# Autodesk Inventor assembly: Robot_V1.0
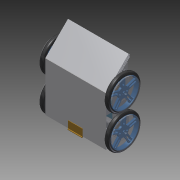
[picture p0: Inventor's stored thumbnail of the model, 180x180]
Saved by Autodesk Inventor 2013 (Build 170138000, 138)
## iProperties
Created: 2015-07-02
Part Number: Robot_V1.0
Document SubType Name: Assembly
Designer: Kyle
Mass: 370.984 g
Surface Area: 2505.11 cm^2
Volume: 171.813 cm^3
Density: 2.15924 g/cm^3
Author: Kyle
## Documents named in this file (16)
- C:\Users\Kyle\Documents\Project documentation\Combat Robot\CAD\V1.0\Robot_V1.0.iam
- C:\Users\Kyle\Documents\Project documentation\Combat Robot\CAD\V1.0\Armor_Rear.iam
- C:\Users\Kyle\Documents\Project documentation\Combat Robot\CAD\V1.0\Armor_Front.iam
- C:\Users\Kyle\Documents\Project documentation\Combat Robot\CAD\V1.0\Gearmotor.iam
- C:\Users\Kyle\Documents\Project documentation\Combat Robot\CAD\V1.0\LiPo.ipt
- C:\Users\Kyle\Documents\Project documentation\Combat Robot\CAD\V1.0\Rx.ipt
- C:\Users\Kyle\Documents\Project documentation\Combat Robot\CAD\V1.0\Plate_InnerSide_Poly.ipt
- C:\Users\Kyle\Documents\Project documentation\Combat Robot\CAD\V1.0\Reinforcer_Front.ipt
- C:\Users\Kyle\Documents\Project documentation\Combat Robot\CAD\V1.0\Bracket.ipt
- C:\Users\Kyle\Documents\Project documentation\Combat Robot\CAD\V1.0\Hinge_Rear.ipt
- C:\Users\Kyle\Documents\Project documentation\Combat Robot\CAD\V1.0\Wheel_60mm.iam
- C:\Users\Kyle\Documents\Project documentation\Combat Robot\CAD\V1.0\Mount_Motor.ipt
- C:\Users\Kyle\Documents\Project documentation\Combat Robot\CAD\V1.0\Bracket_Motor.ipt
- C:\Users\Kyle\Documents\Project documentation\Combat Robot\CAD\V1.0\Plate_Wheel.ipt
- C:\Users\Kyle\Documents\Project documentation\Combat Robot\CAD\V1.0\Plate_Top_Stl22.ipt
- C:\Users\Kyle\Documents\Project documentation\Combat Robot\CAD\V1.0\Chassis_Stl22.ipt
## Components (45 placed, 15 different names)
1. Chassis_Stl22:1 — Mate:24, Mate:45, Flush:34, Flush:35, Flush:36, Flush:37, Mate:51, Mate:52, Mate:78, Flush:44, Mate:79, Flush:45, Mate:81, Flush:46, Mate:83, Flush:47, Mate:85, Mate:88, Mate:97, Angle:1, Angle:2, Angle:3, Angle:4, Mate:171
2. Armor_Rear:1 [sub-assembly] — Mate:24, Mate:46, Mate:49, Flush:36, Flush:37, Mate:50, Mate:53, Mate:87, Mate:90, Mate:92, Mate:95, Mate:98, Mate:153, Mate:167, Flush:58, Mate:170, Flush:59
3. Plate_InnerSide_Poly:1 — Flush:35, Mate:52, Mate:53, Flush:43, Mate:84, Mate:100, Flush:48, Mate:101, Flush:51, Mate:110, Mate:118, Mate:121, Flush:53, Mate:126, Mate:127, Mate:128, Mate:129, Mate:137, Mate:138, Mate:146, Mate:158, Mate:161, Mate:162, Mate:168
4. Plate_InnerSide_Poly:2 — Flush:34, Mate:50, Mate:51, Mate:62, Mate:63, Mate:82, Mate:99, Mate:102, Flush:49, Mate:103, Mate:112, Flush:52, Mate:120, Mate:122, Mate:123, Mate:124, Mate:125, Mate:139, Mate:140, Mate:147, Mate:152, Mate:155, Mate:157, Mate:169, Mate:172
5. Armor_Front:1 [sub-assembly] — Mate:117, Mate:118, Mate:119, Mate:120, Mate:121, Flush:53
6. Plate_Top_Stl22:1 — Flush:43, Mate:104, Mate:105, Flush:50, Mate:106, Mate:107
7. Gearmotor:1 [sub-assembly] — Angle:4, Mate:128, Mate:129, Mate:136, Mate:141, Mate:142, Mate:159, Flush:56
8. Gearmotor:2 [sub-assembly] — Mate:126, Mate:127, Angle:3, Mate:134, Mate:144, Mate:145, Mate:160, Flush:57
9. Gearmotor:3 [sub-assembly] — Angle:1, Mate:122, Mate:123, Mate:130, Mate:150, Mate:151, Mate:154, Flush:54
10. Gearmotor:4 [sub-assembly] — Mate:124, Angle:2, Mate:125, Mate:132, Mate:148, Mate:149, Mate:156, Flush:55
11. LiPo:1 — Mate:45, Mate:46, Mate:48, Mate:62
12. Rx:1 — Mate:48, Mate:49, Mate:63
13. Reinforcer_Front:1 — Mate:117, Mate:171, Mate:172
14. Bracket:1 — Mate:78, Flush:44, Mate:164
15. Bracket:2 — Mate:81, Mate:82, Flush:46
16. Bracket:3 — Mate:88, Mate:90, Mate:91, Mate:93, Mate:165
17. Bracket:4 — Mate:85, Mate:87, Mate:94, Mate:96, Mate:166
18. Bracket:5 — Mate:94, Mate:95, Mate:96
19. Bracket:6 — Mate:97, Mate:98, Mate:99
20. Bracket:7 — Mate:91, Mate:92, Mate:93
21. Bracket:8 — Mate:83, Mate:84, Flush:47
22. Bracket:9 — Mate:79, Flush:45, Mate:163
23. Bracket:10 — Mate:100, Flush:48, Mate:101, Mate:106, Mate:143
24. Bracket:11 — Mate:102, Flush:49, Mate:103, Mate:107
25. Hinge_Rear:1 — Mate:104, Mate:105, Flush:50, Mate:153
26. Bracket:12 — Flush:51, Mate:110, Mate:113, Mate:162, Mate:163
27. Bracket:13 — Mate:112, Flush:52, Mate:113, Mate:119, Mate:164
28. Wheel_60mm:1 [sub-assembly] — Mate:132, Mate:139, Mate:173, Mate:174
29. Wheel_60mm:2 [sub-assembly] — Mate:130, Mate:140, Mate:175, Mate:176
30. Wheel_60mm:3 [sub-assembly] — Mate:136, Mate:138, Mate:177, Mate:178
31. Wheel_60mm:4 [sub-assembly] — Mate:134, Mate:137, Mate:179, Mate:180
32. Mount_Motor:1 — Mate:141, Mate:142, Mate:143
33. Mount_Motor:2 — Mate:144, Mate:145, Mate:146
34. Mount_Motor:3 — Mate:150, Mate:151, Mate:152
35. Mount_Motor:4 — Mate:147, Mate:148, Mate:149
36. Bracket_Motor:1 — Mate:154, Mate:155, Flush:54
37. Bracket_Motor:2 — Mate:156, Mate:157, Flush:55, Mate:165
38. Bracket_Motor:3 — Mate:158, Mate:159, Flush:56
39. Bracket_Motor:4 — Mate:160, Mate:161, Flush:57, Mate:166
40. Bracket:14 — Mate:167, Mate:168, Flush:58
41. Bracket:15 — Mate:169, Mate:170, Flush:59
42. Plate_Wheel:1 — Mate:173, Mate:174
43. Plate_Wheel:2 — Mate:175, Mate:176
44. Plate_Wheel:3 — Mate:179, Mate:180
45. Plate_Wheel:4 — Mate:177, Mate:178
## Relationships (127: Mate 102, Flush 21, Angle 4)
- Mate:24: Chassis_Stl22:1 ↔ Armor_Rear:1
- Mate:45: Chassis_Stl22:1 ↔ LiPo:1
- Mate:46 (12.7 mm): Armor_Rear:1 ↔ LiPo:1
- Mate:48: LiPo:1 ↔ Rx:1
- Mate:49 (12.7 mm): Armor_Rear:1 ↔ Rx:1
- Flush:34: Chassis_Stl22:1 ↔ Plate_InnerSide_Poly:2
- Flush:35: Chassis_Stl22:1 ↔ Plate_InnerSide_Poly:1
- Flush:36: Chassis_Stl22:1 ↔ Armor_Rear:1
- Flush:37: Chassis_Stl22:1 ↔ Armor_Rear:1
- Mate:50: Armor_Rear:1 ↔ Plate_InnerSide_Poly:2
- Mate:51: Chassis_Stl22:1 ↔ Plate_InnerSide_Poly:2
- Mate:52: Chassis_Stl22:1 ↔ Plate_InnerSide_Poly:1
- Mate:53: Armor_Rear:1 ↔ Plate_InnerSide_Poly:1
- Mate:62 (25.4 mm): Plate_InnerSide_Poly:2 ↔ LiPo:1
- Mate:63 (38.1 mm): Plate_InnerSide_Poly:2 ↔ Rx:1
- Flush:43: Plate_InnerSide_Poly:1 ↔ Plate_Top_Stl22:1
- Mate:78: Chassis_Stl22:1 ↔ Bracket:1
- Flush:44 (12.7 mm): Chassis_Stl22:1 ↔ Bracket:1
- Mate:79: Chassis_Stl22:1 ↔ Bracket:9
- Flush:45 (12.7 mm): Chassis_Stl22:1 ↔ Bracket:9
- Mate:81: Chassis_Stl22:1 ↔ Bracket:2
- Mate:82: Plate_InnerSide_Poly:2 ↔ Bracket:2
- Flush:46 (57.15 mm): Chassis_Stl22:1 ↔ Bracket:2
- Mate:83: Chassis_Stl22:1 ↔ Bracket:8
- Mate:84: Plate_InnerSide_Poly:1 ↔ Bracket:8
- Flush:47 (57.15 mm): Chassis_Stl22:1 ↔ Bracket:8
- Mate:85: Chassis_Stl22:1 ↔ Bracket:4
- Mate:87: Armor_Rear:1 ↔ Bracket:4
- Mate:88: Chassis_Stl22:1 ↔ Bracket:3
- Mate:90: Armor_Rear:1 ↔ Bracket:3
- Mate:91: Bracket:3 ↔ Bracket:7
- Mate:92: Armor_Rear:1 ↔ Bracket:7
- Mate:93: Bracket:3 ↔ Bracket:7
- Mate:94: Bracket:4 ↔ Bracket:5
- Mate:95: Armor_Rear:1 ↔ Bracket:5
- Mate:96: Bracket:4 ↔ Bracket:5
- Mate:97: Chassis_Stl22:1 ↔ Bracket:6
- Mate:98: Armor_Rear:1 ↔ Bracket:6
- Mate:99 (48.26 mm): Plate_InnerSide_Poly:2 ↔ Bracket:6
- Mate:100: Plate_InnerSide_Poly:1 ↔ Bracket:10
- Flush:48: Plate_InnerSide_Poly:1 ↔ Bracket:10
- Mate:101 (25.4 mm): Plate_InnerSide_Poly:1 ↔ Bracket:10
- Mate:102: Plate_InnerSide_Poly:2 ↔ Bracket:11
- Flush:49: Plate_InnerSide_Poly:2 ↔ Bracket:11
- Mate:103 (25.4 mm): Plate_InnerSide_Poly:2 ↔ Bracket:11
- Mate:104: Plate_Top_Stl22:1 ↔ Hinge_Rear:1
- Mate:105: Plate_Top_Stl22:1 ↔ Hinge_Rear:1
- Flush:50 (41.91 mm): Plate_Top_Stl22:1 ↔ Hinge_Rear:1
- Mate:106: Plate_Top_Stl22:1 ↔ Bracket:10
- Mate:107: Plate_Top_Stl22:1 ↔ Bracket:11
- Flush:51: Plate_InnerSide_Poly:1 ↔ Bracket:12
- Mate:110 (12.7 mm): Plate_InnerSide_Poly:1 ↔ Bracket:12
- Mate:112: Plate_InnerSide_Poly:2 ↔ Bracket:13
- Flush:52: Plate_InnerSide_Poly:2 ↔ Bracket:13
- Mate:113: Bracket:12 ↔ Bracket:13
- Mate:117: Armor_Front:1 ↔ Reinforcer_Front:1
- Mate:118: Plate_InnerSide_Poly:1 ↔ Armor_Front:1
- Mate:119: Armor_Front:1 ↔ Bracket:13
- Mate:120: Plate_InnerSide_Poly:2 ↔ Armor_Front:1
- Mate:121: Plate_InnerSide_Poly:1 ↔ Armor_Front:1
- Flush:53: Plate_InnerSide_Poly:1 ↔ Armor_Front:1
- Angle:1 (0 deg): Chassis_Stl22:1 ↔ Gearmotor:3
- Mate:122: Plate_InnerSide_Poly:2 ↔ Gearmotor:3
- Mate:123: Plate_InnerSide_Poly:2 ↔ Gearmotor:3
- Mate:124: Plate_InnerSide_Poly:2 ↔ Gearmotor:4
- Angle:2 (0 deg): Chassis_Stl22:1 ↔ Gearmotor:4
- Mate:125: Plate_InnerSide_Poly:2 ↔ Gearmotor:4
- Mate:126: Plate_InnerSide_Poly:1 ↔ Gearmotor:2
- Mate:127: Plate_InnerSide_Poly:1 ↔ Gearmotor:2
- Angle:3 (0 deg): Chassis_Stl22:1 ↔ Gearmotor:2
- Angle:4 (0 deg): Chassis_Stl22:1 ↔ Gearmotor:1
- Mate:128: Plate_InnerSide_Poly:1 ↔ Gearmotor:1
- Mate:129: Plate_InnerSide_Poly:1 ↔ Gearmotor:1
- Mate:130: Gearmotor:3 ↔ Wheel_60mm:2
- Mate:132: Gearmotor:4 ↔ Wheel_60mm:1
- Mate:134: Gearmotor:2 ↔ Wheel_60mm:4
- Mate:136: Gearmotor:1 ↔ Wheel_60mm:3
- Mate:137: Plate_InnerSide_Poly:1 ↔ Wheel_60mm:4
- Mate:138: Plate_InnerSide_Poly:1 ↔ Wheel_60mm:3
- Mate:139: Plate_InnerSide_Poly:2 ↔ Wheel_60mm:1
- Mate:140: Plate_InnerSide_Poly:2 ↔ Wheel_60mm:2
- Mate:141: Gearmotor:1 ↔ Mount_Motor:1
- Mate:142: Gearmotor:1 ↔ Mount_Motor:1
- Mate:143: Bracket:10 ↔ Mount_Motor:1
- Mate:144: Gearmotor:2 ↔ Mount_Motor:2
- Mate:145: Gearmotor:2 ↔ Mount_Motor:2
- Mate:146: Plate_InnerSide_Poly:1 ↔ Mount_Motor:2
- Mate:147: Plate_InnerSide_Poly:2 ↔ Mount_Motor:4
- Mate:148: Gearmotor:4 ↔ Mount_Motor:4
- Mate:149: Gearmotor:4 ↔ Mount_Motor:4
- Mate:150: Gearmotor:3 ↔ Mount_Motor:3
- Mate:151: Gearmotor:3 ↔ Mount_Motor:3
- Mate:152: Plate_InnerSide_Poly:2 ↔ Mount_Motor:3
- Mate:153: Armor_Rear:1 ↔ Hinge_Rear:1
- Mate:154: Gearmotor:3 ↔ Bracket_Motor:1
- Mate:155: Plate_InnerSide_Poly:2 ↔ Bracket_Motor:1
- Flush:54 (6.35 mm): Gearmotor:3 ↔ Bracket_Motor:1
- Mate:156: Gearmotor:4 ↔ Bracket_Motor:2
- Mate:157: Plate_InnerSide_Poly:2 ↔ Bracket_Motor:2
- Flush:55 (-6.35 mm): Gearmotor:4 ↔ Bracket_Motor:2
- Mate:158: Plate_InnerSide_Poly:1 ↔ Bracket_Motor:3
- Mate:159: Gearmotor:1 ↔ Bracket_Motor:3
- Flush:56 (6.35 mm): Gearmotor:1 ↔ Bracket_Motor:3
- Mate:160: Gearmotor:2 ↔ Bracket_Motor:4
- Mate:161: Plate_InnerSide_Poly:1 ↔ Bracket_Motor:4
- Flush:57 (6.35 mm): Gearmotor:2 ↔ Bracket_Motor:4
- Mate:162: Plate_InnerSide_Poly:1 ↔ Bracket:12
- Mate:163: Bracket:9 ↔ Bracket:12
- Mate:164: Bracket:1 ↔ Bracket:13
- Mate:165: Bracket:3 ↔ Bracket_Motor:2
- Mate:166: Bracket:4 ↔ Bracket_Motor:4
- Mate:167: Armor_Rear:1 ↔ Bracket:14
- Mate:168: Plate_InnerSide_Poly:1 ↔ Bracket:14
- Flush:58: Armor_Rear:1 ↔ Bracket:14
- Mate:169: Plate_InnerSide_Poly:2 ↔ Bracket:15
- Mate:170: Armor_Rear:1 ↔ Bracket:15
- Flush:59: Armor_Rear:1 ↔ Bracket:15
- Mate:171: Chassis_Stl22:1 ↔ Reinforcer_Front:1
- Mate:172 (47.0916 mm): Plate_InnerSide_Poly:2 ↔ Reinforcer_Front:1
- Mate:173: Wheel_60mm:1 ↔ Plate_Wheel:1
- Mate:174: Wheel_60mm:1 ↔ Plate_Wheel:1
- Mate:175: Wheel_60mm:2 ↔ Plate_Wheel:2
- Mate:176: Wheel_60mm:2 ↔ Plate_Wheel:2
- Mate:177: Wheel_60mm:3 ↔ Plate_Wheel:4
- Mate:178: Wheel_60mm:3 ↔ Plate_Wheel:4
- Mate:179: Wheel_60mm:4 ↔ Plate_Wheel:3
- Mate:180: Wheel_60mm:4 ↔ Plate_Wheel:3
